# Autodesk Inventor assembly: display_mit_pi
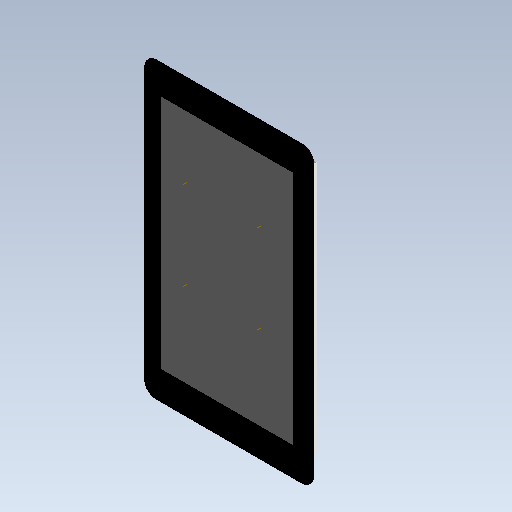
[picture p0: Inventor's stored thumbnail of the model, 512x512]
Saved by Autodesk Inventor 2021 (Build 250183000, 183)
## iProperties
Created: 2021-07-20
Part Number: display_mit_pi
Document SubType Name: Assembly
Designer: Simon
Author: Simon
## Documents named in this file (4)
- C:\WORK\MILK_COOLER\display_mit_pi.iam
- C:\WORK\MILK_COOLER\display.ipt
- C:\WORK\MILK_COOLER\raspberrypi\Raspberry Pi 3.iam
- C:\Users\simub\Documents\Inventor\Content Center Files\R2021\de-DE\AS 1427(01)\AS 1427 - M2.5 x 10(3).ipt
## Components (6 placed, 3 different names)
1. display:1 — Fluchtend:1, Fluchtend:2, Fluchtend:3, Passend:1, Passend:2, Passend:3
2. Raspberry Pi 3:1 [sub-assembly] — Passend:1, Passend:2, Passend:3, Einfügen:1, Einfügen:2, Einfügen:3, Einfügen:4
3. AS 1427 - Metrisch M2.5 x 10:1 — Einfügen:4
4. AS 1427 - Metrisch M2.5 x 10:2 — Einfügen:3
5. AS 1427 - Metrisch M2.5 x 10:3 — Einfügen:2
6. AS 1427 - Metrisch M2.5 x 10:4 — Einfügen:1
## Relationships (10: Insert 4, Flush 3, Mate 3)
- Fluchtend:1 [Flush]: display:1
- Fluchtend:2 [Flush]: display:1
- Fluchtend:3 [Flush]: display:1
- Passend:1 [Mate]: display:1 ↔ Raspberry Pi 3:1
- Passend:2 [Mate]: display:1 ↔ Raspberry Pi 3:1
- Passend:3 [Mate]: display:1 ↔ Raspberry Pi 3:1
- Einfügen:1 [Insert]: Raspberry Pi 3:1 ↔ AS 1427 - Metrisch M2.5 x 10:4
- Einfügen:2 [Insert]: Raspberry Pi 3:1 ↔ AS 1427 - Metrisch M2.5 x 10:3
- Einfügen:3 [Insert]: Raspberry Pi 3:1 ↔ AS 1427 - Metrisch M2.5 x 10:2
- Einfügen:4 [Insert]: Raspberry Pi 3:1 ↔ AS 1427 - Metrisch M2.5 x 10:1
